# Autodesk Inventor assembly: Roller_Bracket
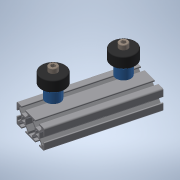
[picture p0: Inventor's stored thumbnail of the model, 180x180]
Saved by Autodesk Inventor 2021 (Build 250183000, 183)
## iProperties
Created: 2021-02-01
Part Number: Roller_Bracket
Document SubType Name: Assembly
Designer: Jorian Brusind
Mass: 44.0669 g
Surface Area: 169.812 cm^2
Volume: 42.4218 cm^3
Density: 1.03878 g/cm^3
Author: Jorian Brusind
## Documents named in this file (5)
- C:\Users\Jorian Brusind\Documents\GitHub\PersonalProjects\HyperRail\Inventor Files\Roller_Bracket.iam
- C:\Users\Jorian Brusind\Documents\GitHub\PersonalProjects\HyperRail\Inventor Files\11mm_BearingWheel.ipt
- C:\Users\Jorian Brusind\Documents\GitHub\PersonalProjects\Inventor Projects\Useful models\8020_Sets\IPT_20_Series\IPT_20_Series\20-2040_150mm.ipt
- C:\Users\Jorian Brusind\Documents\GitHub\PersonalProjects\HyperRail\Inventor Files\4mm_Roller_Spacer.ipt
- C:\Users\Jorian Brusind\Documents\GitHub\PersonalProjects\Inventor Projects\Useful models\Metric bolt\Bolt M5 30mm.ipt
## Components (7 placed, 4 different names)
1. 11mm_BearingWheel:1 — Mate:21, Mate:22, Mate:29
2. 11mm_BearingWheel:2 — Mate:20, Mate:23, Mate:24, Mate:26
3. 20-2040_150mm:1 — Mate:20, Mate:27, Mate:30, Mate:31, Mate:32, Mate:33
4. 4mm_Roller_Spacer:1 — Mate:25, Mate:26, Mate:27, Mate:32
5. 4mm_Roller_Spacer:2 — Mate:28, Mate:29, Mate:30, Mate:31, Mate:33
6. Bolt M5 30mm:1 — Mate:21, Mate:22, Mate:28
7. Bolt M5 30mm:2 — Mate:23, Mate:24, Mate:25
## Relationships (14: Mate 14)
- Mate:20 (-16 mm): 11mm_BearingWheel:2 ↔ 20-2040_150mm:1
- Mate:21: 11mm_BearingWheel:1 ↔ Bolt M5 30mm:1
- Mate:22: 11mm_BearingWheel:1 ↔ Bolt M5 30mm:1
- Mate:23: 11mm_BearingWheel:2 ↔ Bolt M5 30mm:2
- Mate:24: 11mm_BearingWheel:2 ↔ Bolt M5 30mm:2
- Mate:25: 4mm_Roller_Spacer:1 ↔ Bolt M5 30mm:2
- Mate:26: 11mm_BearingWheel:2 ↔ 4mm_Roller_Spacer:1
- Mate:27: 20-2040_150mm:1 ↔ 4mm_Roller_Spacer:1
- Mate:28: 4mm_Roller_Spacer:2 ↔ Bolt M5 30mm:1
- Mate:29: 11mm_BearingWheel:1 ↔ 4mm_Roller_Spacer:2
- Mate:30: 20-2040_150mm:1 ↔ 4mm_Roller_Spacer:2
- Mate:31 (2.75 mm): 20-2040_150mm:1 ↔ 4mm_Roller_Spacer:2
- Mate:32 (2.75 mm): 20-2040_150mm:1 ↔ 4mm_Roller_Spacer:1
- Mate:33 (-25 mm): 20-2040_150mm:1 ↔ 4mm_Roller_Spacer:2
